# Autodesk Inventor assembly: СБ_Инфотабло
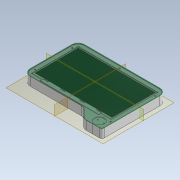
[picture p0: Inventor's stored thumbnail of the model, 180x180]
Saved by Autodesk Inventor 2021.2 (Build 252289000, 289)
## iProperties
Created: 2022-11-28
Part Number: СБ_Инфотабло
Document SubType Name: Assembly
Designer: Voodoo
Mass: 1593.93 g
Surface Area: 12220.1 cm^2
Volume: 1576.45 cm^3
Density: 1.01109 g/cm^3
Author: Voodoo
## Documents named in this file (21)
- C:\Users\Voodoo\Documents\Inventor\АБТ_Инфотабло\СБ_Инфотабло.iam
- C:\Users\Voodoo\Documents\Inventor\АБТ_Инфотабло\NV173FHM-N4G V8.0.ipt
- C:\Users\Voodoo\Documents\Inventor\АБТ_Инфотабло\Блок питания LS-50-5_5V.ipt
- C:\Users\Voodoo\Documents\Inventor\АБТ_Инфотабло\Блок питания MA-60-12_12V.ipt
- C:\Users\Voodoo\Documents\Inventor\АБТ_Инфотабло\Медиа приставка GIBORIY X96 Mini 2.ipt
- C:\Users\Voodoo\Documents\Inventor\АБТ_Инфотабло\Обечайка часть 1.ipt
- C:\Users\Voodoo\Documents\Inventor\АБТ_Инфотабло\Обечайка часть 2.ipt
- C:\Users\Voodoo\Documents\Inventor\АБТ_Инфотабло\Лицевой лист.ipt
- C:\Users\Voodoo\Documents\Inventor\АБТ_Инфотабло\Монтажный лист.ipt
- C:\Users\Voodoo\Documents\Inventor\АБТ_Инфотабло\Вытяжная заклепка_Р-Ш-М3-Ум.ipt
- C:\Users\Voodoo\Documents\Inventor\АБТ_Инфотабло\Скоба БП1.ipt
- C:\Users\Voodoo\Documents\Inventor\АБТ_Инфотабло\Скоба БП2.ipt
- C:\Users\Voodoo\Documents\Inventor\АБТ_Инфотабло\Кронштейн медиа приставки.ipt
- C:\Users\Voodoo\Documents\Inventor\Content Center Files\R2021\Metizi\Shp_3x8.ipt
- C:\Users\Voodoo\Documents\Inventor\АБТ_Инфотабло\Короб задний.ipt
- C:\Users\Voodoo\Documents\Inventor\Content Center Files\R2021\Metizi\PEM_S_M5_1.ipt
- C:\Users\Voodoo\Documents\Inventor\Content Center Files\R2021\Metizi\Shp_4x8.ipt
- C:\Users\Voodoo\Documents\Inventor\АБТ_Инфотабло\Стекло.ipt
- C:\Users\Voodoo\Documents\Inventor\Content Center Files\R2021\ru-RU\AS 1427(05)\AS 1427 - M3 x 6(5) II.ipt
- C:\Users\Voodoo\Documents\Inventor\Content Center Files\R2021\ru-RU\ANSI B18.2.4.2M\ANSI B18.2.4.2M - M3x0,5 - 5,5.ipt
- C:\Users\Voodoo\Documents\Inventor\АБТ_Инфотабло\Плата контроллера.ipt
## Components (49 placed, 20 different names)
1. NV173FHM-N4G V8.0:1 — Заподлицо:17, Совмещение:36, Совмещение:37
2. Медиа приставка GIBORIY X96 Mini 2:1 — Совмещение:55, Совмещение:56, Совмещение:57
3. Обечайка часть 1:1 — Заподлицо:10, Совмещение:4, Заподлицо:11, Совмещение:31, Заподлицо:20, Совмещение:59
4. Обечайка часть 2:1 — Заподлицо:7, Заподлицо:8, Заподлицо:9, Заподлицо:10, Совмещение:4, Заподлицо:11, Заподлицо:16, Совмещение:32, Совмещение:44, Заподлицо:21, Совмещение:51, Совмещение:58, Совмещение:67, Совмещение:69
5. Лицевой лист:1 — Заподлицо:16, Совмещение:31, Совмещение:32, Совмещение:33, Совмещение:34, Совмещение:35, Вставка:16, Вставка:17, Вставка:18, Вставка:19, Вставка:20, Заподлицо:17, Совмещение:36, Совмещение:37
6. Монтажный лист:1 — Совмещение:33, Совмещение:34, Совмещение:35, Вставка:21, Вставка:22, Вставка:23, Вставка:24, Вставка:25, Вставка:26, Вставка:27, Вставка:28, Вставка:29, Вставка:30, Совмещение:40, Совмещение:42, Совмещение:43, Вставка:31, Вставка:32, Вставка:33, Совмещение:55, Совмещение:60, Совмещение:62, Совмещение:63, Вставка:43, Вставка:44, Вставка:45, Вставка:46, Совмещение:70, Совмещение:72
7. Вытяжная заклепка_Р-Ш-М3-Ум:1 — Вставка:19, Вставка:40
8. Вытяжная заклепка_Р-Ш-М3-Ум:2 — Вставка:17, Вставка:42
9. Вытяжная заклепка_Р-Ш-М3-Ум:3 — Вставка:16, Вставка:38
10. Вытяжная заклепка_Р-Ш-М3-Ум:4 — Вставка:20, Вставка:39
11. Вытяжная заклепка_Р-Ш-М3-Ум:5 — Вставка:18, Вставка:41
12. Скоба БП1:1 — Совмещение:42, Совмещение:61, Заподлицо:22, Совмещение:65
13. Скоба БП2:1 — Совмещение:40, Совмещение:64, Заподлицо:23, Совмещение:65
14. Shp_3x8:1 — Вставка:29
15. Shp_3x8:2 — Вставка:24
16. Shp_3x8:3 — Вставка:26
17. Shp_3x8:4 — Вставка:23
18. Shp_3x8:5 — Вставка:22
19. Shp_3x8:6 — Вставка:25
20. Короб задний:1 — Заподлицо:15, Вставка:12, Вставка:13, Вставка:14, Вставка:15, Совмещение:43, Совмещение:44, Вставка:34, Вставка:35, Вставка:36, Вставка:37
21. PEM_S_M5_1:1 — Вставка:14
22. PEM_S_M5_1:2 — Вставка:13
23. PEM_S_M5_1:3 — Вставка:12
24. PEM_S_M5_1:4 — Вставка:15
25. Shp_4x8:1 — Вставка:28
26. Shp_4x8:2 — Вставка:21
27. Shp_4x8:3 — Вставка:27
28. Shp_4x8:4 — Вставка:30
29. Стекло:1 — Заподлицо:20, Заподлицо:21, Совмещение:51
30. Shp_3x8:7 — Вставка:31
31. Shp_3x8:8 — Вставка:32
32. Shp_3x8:9 — Вставка:33
33. AS 1427 H - метрическая M3 x 6:1 — Вставка:41
34. AS 1427 H - метрическая M3 x 6:2 — Вставка:42
35. AS 1427 H - метрическая M3 x 6:3 — Вставка:39
36. AS 1427 H - метрическая M3 x 6:4 — Вставка:40
37. AS 1427 H - метрическая M3 x 6:5 — Вставка:38
38. ANSI B18.2.4.2M M3x0,5:1 — Вставка:34
39. ANSI B18.2.4.2M M3x0,5:2 — Вставка:35
40. ANSI B18.2.4.2M M3x0,5:3 — Вставка:36
41. ANSI B18.2.4.2M M3x0,5:4 — Вставка:37
42. Блок питания LS-50-5_5V:2 — Совмещение:63, Совмещение:64, Заподлицо:23, Совмещение:68, Совмещение:69
43. Блок питания MA-60-12_12V:2 — Совмещение:61, Совмещение:62, Заподлицо:22, Совмещение:67, Совмещение:68
44. Кронштейн медиа приставки:2 — Совмещение:56, Совмещение:57, Совмещение:58, Совмещение:59, Совмещение:60
45. Shp_3x8:10 — Вставка:44, Совмещение:72
46. Shp_3x8:11 — Вставка:43, Совмещение:71
47. Shp_3x8:12 — Вставка:45
48. Shp_3x8:13 — Вставка:46
49. Плата контроллера:1 — Совмещение:70, Совмещение:71
## Relationships (77: Insert 35, Mate 30, Flush 12)
- Заподлицо:7 [Flush]: Обечайка часть 2:1
- Заподлицо:8 [Flush]: Обечайка часть 2:1
- Заподлицо:9 [Flush]: Обечайка часть 2:1
- Заподлицо:10 [Flush]: Обечайка часть 1:1 ↔ Обечайка часть 2:1
- Совмещение:4 [Mate]: Обечайка часть 1:1 ↔ Обечайка часть 2:1
- Заподлицо:11 [Flush]: Обечайка часть 1:1 ↔ Обечайка часть 2:1
- Заподлицо:15 [Flush]: Короб задний:1
- Вставка:12 [Insert]: Короб задний:1 ↔ PEM_S_M5_1:3
- Вставка:13 [Insert]: Короб задний:1 ↔ PEM_S_M5_1:2
- Вставка:14 [Insert]: Короб задний:1 ↔ PEM_S_M5_1:1
- Вставка:15 [Insert]: Короб задний:1 ↔ PEM_S_M5_1:4
- Заподлицо:16 [Flush] (2 mm): Обечайка часть 2:1 ↔ Лицевой лист:1
- Совмещение:31 [Mate]: Обечайка часть 1:1 ↔ Лицевой лист:1
- Совмещение:32 [Mate]: Обечайка часть 2:1 ↔ Лицевой лист:1
- Совмещение:33 [Mate]: Лицевой лист:1 ↔ Монтажный лист:1
- Совмещение:34 [Mate]: Лицевой лист:1 ↔ Монтажный лист:1
- Совмещение:35 [Mate]: Лицевой лист:1 ↔ Монтажный лист:1
- Вставка:16 [Insert]: Лицевой лист:1 ↔ Вытяжная заклепка_Р-Ш-М3-Ум:3
- Вставка:17 [Insert]: Лицевой лист:1 ↔ Вытяжная заклепка_Р-Ш-М3-Ум:2
- Вставка:18 [Insert]: Лицевой лист:1 ↔ Вытяжная заклепка_Р-Ш-М3-Ум:5
- Вставка:19 [Insert]: Лицевой лист:1 ↔ Вытяжная заклепка_Р-Ш-М3-Ум:1
- Вставка:20 [Insert]: Лицевой лист:1 ↔ Вытяжная заклепка_Р-Ш-М3-Ум:4
- Вставка:21 [Insert]: Монтажный лист:1 ↔ Shp_4x8:2
- Вставка:22 [Insert]: Монтажный лист:1 ↔ Shp_3x8:5
- Вставка:23 [Insert]: Монтажный лист:1 ↔ Shp_3x8:4
- Вставка:24 [Insert]: Монтажный лист:1 ↔ Shp_3x8:2
- Вставка:25 [Insert]: Монтажный лист:1 ↔ Shp_3x8:6
- Вставка:26 [Insert]: Монтажный лист:1 ↔ Shp_3x8:3
- Вставка:27 [Insert]: Монтажный лист:1 ↔ Shp_4x8:3
- Вставка:28 [Insert]: Монтажный лист:1 ↔ Shp_4x8:1
- Вставка:29 [Insert]: Монтажный лист:1 ↔ Shp_3x8:1
- Вставка:30 [Insert]: Монтажный лист:1 ↔ Shp_4x8:4
- Заподлицо:17 [Flush]: NV173FHM-N4G V8.0:1 ↔ Лицевой лист:1
- Совмещение:36 [Mate] (3 mm): NV173FHM-N4G V8.0:1 ↔ Лицевой лист:1
- Совмещение:37 [Mate] (3 mm): NV173FHM-N4G V8.0:1 ↔ Лицевой лист:1
- Совмещение:40 [Mate]: Монтажный лист:1 ↔ Скоба БП2:1
- Совмещение:42 [Mate]: Монтажный лист:1 ↔ Скоба БП1:1
- Совмещение:43 [Mate]: Монтажный лист:1 ↔ Короб задний:1
- Совмещение:44 [Mate] (18 mm): Обечайка часть 2:1 ↔ Короб задний:1
- Заподлицо:20 [Flush]: Обечайка часть 1:1 ↔ Стекло:1
- Заподлицо:21 [Flush]: Обечайка часть 2:1 ↔ Стекло:1
- Совмещение:51 [Mate]: Обечайка часть 2:1 ↔ Стекло:1
- Вставка:31 [Insert]: Монтажный лист:1 ↔ Shp_3x8:7
- Вставка:32 [Insert]: Монтажный лист:1 ↔ Shp_3x8:8
- Вставка:33 [Insert]: Монтажный лист:1 ↔ Shp_3x8:9
- Вставка:34 [Insert]: Короб задний:1 ↔ ANSI B18.2.4.2M M3x0,5:1
- Вставка:35 [Insert]: Короб задний:1 ↔ ANSI B18.2.4.2M M3x0,5:2
- Вставка:36 [Insert]: Короб задний:1 ↔ ANSI B18.2.4.2M M3x0,5:3
- Вставка:37 [Insert]: Короб задний:1 ↔ ANSI B18.2.4.2M M3x0,5:4
- Вставка:38 [Insert]: Вытяжная заклепка_Р-Ш-М3-Ум:3 ↔ AS 1427 H - метрическая M3 x 6:5
- Вставка:39 [Insert]: Вытяжная заклепка_Р-Ш-М3-Ум:4 ↔ AS 1427 H - метрическая M3 x 6:3
- Вставка:40 [Insert]: Вытяжная заклепка_Р-Ш-М3-Ум:1 ↔ AS 1427 H - метрическая M3 x 6:4
- Вставка:41 [Insert]: Вытяжная заклепка_Р-Ш-М3-Ум:5 ↔ AS 1427 H - метрическая M3 x 6:1
- Вставка:42 [Insert]: Вытяжная заклепка_Р-Ш-М3-Ум:2 ↔ AS 1427 H - метрическая M3 x 6:2
- Совмещение:55 [Mate]: Медиа приставка GIBORIY X96 Mini 2:1 ↔ Монтажный лист:1
- Совмещение:56 [Mate] (1 mm): Медиа приставка GIBORIY X96 Mini 2:1 ↔ Кронштейн медиа приставки:2
- Совмещение:57 [Mate] (1 mm): Медиа приставка GIBORIY X96 Mini 2:1 ↔ Кронштейн медиа приставки:2
- Совмещение:58 [Mate] (40 mm): Обечайка часть 2:1 ↔ Кронштейн медиа приставки:2
- Совмещение:59 [Mate] (50 mm): Обечайка часть 1:1 ↔ Кронштейн медиа приставки:2
- Совмещение:60 [Mate]: Монтажный лист:1 ↔ Кронштейн медиа приставки:2
- Совмещение:61 [Mate]: Скоба БП1:1 ↔ Блок питания MA-60-12_12V:2
- Совмещение:62 [Mate]: Монтажный лист:1 ↔ Блок питания MA-60-12_12V:2
- Заподлицо:22 [Flush] (50 mm): Скоба БП1:1 ↔ Блок питания MA-60-12_12V:2
- Совмещение:63 [Mate]: Монтажный лист:1 ↔ Блок питания LS-50-5_5V:2
- Совмещение:64 [Mate] (0.5 mm): Скоба БП2:1 ↔ Блок питания LS-50-5_5V:2
- Заподлицо:23 [Flush] (35 mm): Скоба БП2:1 ↔ Блок питания LS-50-5_5V:2
- Совмещение:65 [Mate] (5 mm): Скоба БП1:1 ↔ Скоба БП2:1
- Совмещение:67 [Mate] (40 mm): Обечайка часть 2:1 ↔ Блок питания MA-60-12_12V:2
- Совмещение:68 [Mate] (20 mm): Блок питания LS-50-5_5V:2 ↔ Блок питания MA-60-12_12V:2
- Совмещение:69 [Mate] (60 mm): Обечайка часть 2:1 ↔ Блок питания LS-50-5_5V:2
- Вставка:43 [Insert]: Монтажный лист:1 ↔ Shp_3x8:11
- Вставка:44 [Insert]: Монтажный лист:1 ↔ Shp_3x8:10
- Вставка:45 [Insert]: Монтажный лист:1 ↔ Shp_3x8:12
- Вставка:46 [Insert]: Монтажный лист:1 ↔ Shp_3x8:13
- Совмещение:70 [Mate]: Монтажный лист:1 ↔ Плата контроллера:1
- Совмещение:71 [Mate]: Shp_3x8:11 ↔ Плата контроллера:1
- Совмещение:72 [Mate]: Монтажный лист:1 ↔ Shp_3x8:10
